# Autodesk Inventor assembly: toe
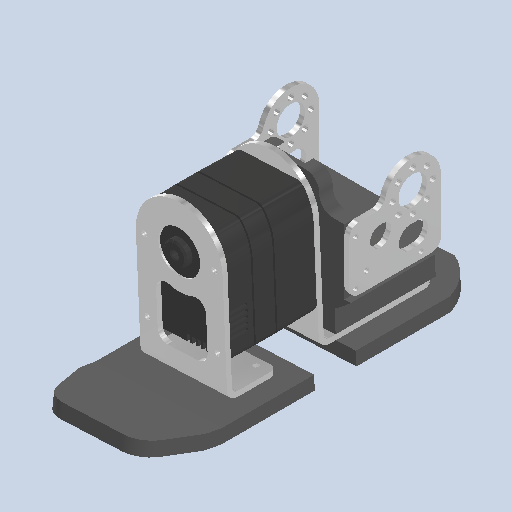
[picture p0: Inventor's stored thumbnail of the model, 512x512]
Saved by Autodesk Inventor 2026.1 (Build 301233020, 233B)
## iProperties
Created: 2024-02-12
Part Number: toe
Document SubType Name: Assembly
Designer: hibik
Author: hibik
## Documents named in this file (9)
- C:\Users\hibik\Documents\Robomech\HR\Eglantyne_mark2\hard\leg\toe.iam
- C:\Users\hibik\Documents\Robomech\HR\Eglantyne_mark2\hard\leg\toe_joint.iam
- C:\Users\hibik\Documents\Robomech\HR\Eglantyne_mark2\hard\leg\toe_back.ipt
- C:\Users\hibik\Desktop\ロボメカ\HR\2024.02.11 Rl\KRS3300サーボホーン.ipt
- C:\Users\hibik\Desktop\ロボメカ\HR\2024.02.11 Rl\KRS3300モータ.ipt
- C:\Users\hibik\Documents\Robomech\HR\Eglantyne_mark2\hard\leg\toe_front.ipt
- C:\Users\hibik\Documents\Robomech\HR\Eglantyne_mark2\hard\leg\toe_back_buf.ipt
- C:\Users\hibik\Documents\Robomech\HR\Eglantyne_mark2\hard\leg\toe_sole_front_big.ipt
- C:\Users\hibik\Documents\Robomech\HR\Eglantyne_mark2\hard\leg\toe_sole_bac_big.ipt
## Components (8 placed, 8 different names)
1. toe_joint:1 [sub-assembly] — 挿入:4, 挿入:9
2. toe_back:1 — メイト:1, 挿入:1, 角度:1, メイト:3, フラッシュ:1, フラッシュ:2, 角度:2
3. KRS3300サーボホーン:2 — 挿入:3, 挿入:4, 挿入:9
4. KRS3300モータ:1 — メイト:1, 挿入:1, 角度:1, 挿入:3, メイト:2, 挿入:6
5. toe_front:1 — メイト:2, 挿入:6, 角度:2, 挿入:10, 挿入:11
6. toe_back_buf:1 — メイト:3, フラッシュ:1, フラッシュ:2, 挿入:12, 挿入:13
7. toe_sole_front_big:1 — 挿入:10, 挿入:11
8. toe_sole_bac_big:1 — 挿入:12, 挿入:13
## Relationships (16: Insert 9, Mate 3, Angle 2, Flush 2)
- メイト:1 [Mate]: toe_back:1 ↔ KRS3300モータ:1
- 挿入:1 [Insert]: toe_back:1 ↔ KRS3300モータ:1
- 角度:1 [Angle] (0 deg): toe_back:1 ↔ KRS3300モータ:1
- 挿入:3 [Insert] (0.3 mm): KRS3300サーボホーン:2 ↔ KRS3300モータ:1
- 挿入:4 [Insert]: toe_joint:1 ↔ KRS3300サーボホーン:2
- メイト:2 [Mate]: KRS3300モータ:1 ↔ toe_front:1
- 挿入:6 [Insert]: KRS3300モータ:1 ↔ toe_front:1
- メイト:3 [Mate]: toe_back:1 ↔ toe_back_buf:1
- フラッシュ:1 [Flush]: toe_back:1 ↔ toe_back_buf:1
- フラッシュ:2 [Flush]: toe_back:1 ↔ toe_back_buf:1
- 角度:2 [Angle] (0 deg): toe_back:1 ↔ toe_front:1
- 挿入:9 [Insert]: toe_joint:1 ↔ KRS3300サーボホーン:2
- 挿入:10 [Insert]: toe_front:1 ↔ toe_sole_front_big:1
- 挿入:11 [Insert]: toe_front:1 ↔ toe_sole_front_big:1
- 挿入:12 [Insert] (1.5 mm): toe_back_buf:1 ↔ toe_sole_bac_big:1
- 挿入:13 [Insert] (1.5 mm): toe_back_buf:1 ↔ toe_sole_bac_big:1
